# Autodesk Inventor assembly: base-frame
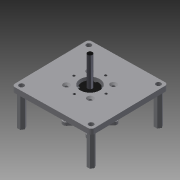
[picture p0: Inventor's stored thumbnail of the model, 180x180]
Saved by Autodesk Inventor 2015 (Build 190159000, 159)
## iProperties
Created: 2015-12-01
Part Number: base-frame
Document SubType Name: Assembly
Designer: jufranz
Author: jufranz
## Documents named in this file (6)
- \\engin-labs.m.storage.umich.edu\jufranz\windat.V2\Documents\Inventor\perspection\base-frame.iam
- \\engin-labs.m.storage.umich.edu\jufranz\windat.V2\Documents\Inventor\perspection\base_mount.ipt
- \\engin-labs.m.storage.umich.edu\jufranz\windat.V2\Documents\Inventor\perspection\standoff.ipt
- \\engin-labs.m.storage.umich.edu\jufranz\windat.V2\Documents\Inventor\perspection\Imported Components\motor_base\motor_base.ipt
- \\engin-labs.m.storage.umich.edu\jufranz\windat.V2\Documents\Inventor\perspection\Imported Components\Tiger-Motor\Tiger-Motor.iam
- \\engin-labs.m.storage.umich.edu\jufranz\windat.V2\Documents\Inventor\perspection\standoff_m5.ipt
## Components (11 placed, 5 different names)
1. base_mount:1 — Insert:1, Insert:2, Insert:3, Insert:4, Insert:9, Insert:10, Insert:11, Insert:12
2. standoff:1 — Insert:1, Insert:5
3. standoff:2 — Insert:2
4. standoff:3 — Insert:3
5. standoff:4 — Insert:4, Insert:6
6. motor_base:1 — Insert:5, Insert:6, Insert:7, Insert:8
7. Tiger-Motor:1 [sub-assembly] — Insert:7, Insert:8
8. standoff_m5:1 — Insert:9
9. standoff_m5:2 — Insert:10
10. standoff_m5:3 — Insert:11
11. standoff_m5:4 — Insert:12
## Relationships (12: Insert 12)
- Insert:1: base_mount:1 ↔ standoff:1
- Insert:2: base_mount:1 ↔ standoff:2
- Insert:3: base_mount:1 ↔ standoff:3
- Insert:4: base_mount:1 ↔ standoff:4
- Insert:5: standoff:1 ↔ motor_base:1
- Insert:6: standoff:4 ↔ motor_base:1
- Insert:7: motor_base:1 ↔ Tiger-Motor:1
- Insert:8: motor_base:1 ↔ Tiger-Motor:1
- Insert:9: base_mount:1 ↔ standoff_m5:1
- Insert:10: base_mount:1 ↔ standoff_m5:2
- Insert:11: base_mount:1 ↔ standoff_m5:3
- Insert:12: base_mount:1 ↔ standoff_m5:4
